# Autodesk Inventor assembly: Wheel_60mm
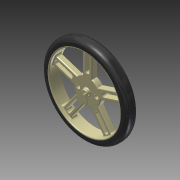
[picture p0: Inventor's stored thumbnail of the model, 180x180]
Saved by Autodesk Inventor 2013 (Build 170138000, 138)
## iProperties
Created: 2015-07-06
Part Number: Wheel_60mm
Document SubType Name: Assembly
Designer: Kyle
Mass: 10.7351 g
Surface Area: 90.1972 cm^2
Volume: 8.91864 cm^3
Density: 1.20367 g/cm^3
Author: Kyle
## Documents named in this file (3)
- C:\Users\Kyle\Documents\Project documentation\Combat Robot\CAD\V1.0\Wheel_60mm.iam
- C:\Users\Kyle\Documents\Project documentation\Combat Robot\CAD\V1.0\Wheel_Rim.ipt
- C:\Users\Kyle\Documents\Project documentation\Combat Robot\CAD\V1.0\Wheel_Tire.ipt
## Components (2 placed, 2 different names)
1. Wheel_Rim:1 — Mate:1, Mate:2
2. Wheel_Tire:1 — Mate:1, Mate:2
## Relationships (2: Mate 2)
- Mate:1: Wheel_Rim:1 ↔ Wheel_Tire:1
- Mate:2: Wheel_Rim:1 ↔ Wheel_Tire:1
